# Autodesk Inventor assembly: Cylinder_Printer
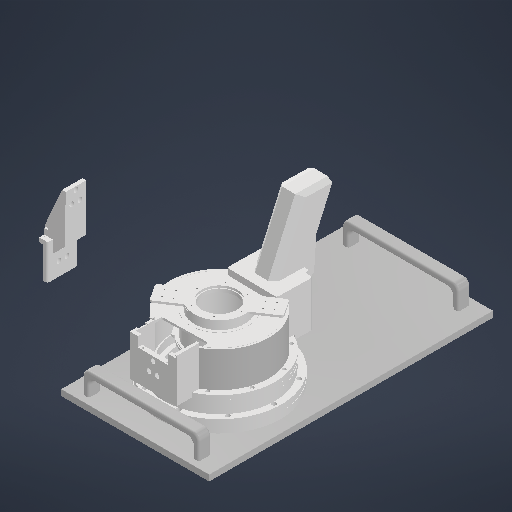
[picture p0: Inventor's stored thumbnail of the model, 512x512]
Saved by Autodesk Inventor 2026 (Build 300175000, 175)
## iProperties
Created: 2025-05-09
Part Number: Cylinder_Printer
Document SubType Name: Assembly
Designer: Charl
Author: Charl
## Documents named in this file (3)
- C:\School\Research\Inventor\v0.2.2\ASM\Cylinder_Printer.iam
- C:\School\Research\Inventor\v0.2.2\ASM\Cylinder_Cover_ASM.iam
- C:\School\Research\Inventor\v0.2.2\ASM\Printer\Cover.ipt
## Components (2 placed, 2 different names)
1. Cylinder_Cover_ASM:1 [sub-assembly] — Mate:1, Mate:2
2. Cover:1 — Mate:1, Mate:2
## Relationships (2: Mate 2)
- Mate:1: Cylinder_Cover_ASM:1 ↔ Cover:1
- Mate:2: Cylinder_Cover_ASM:1 ↔ Cover:1
